# Autodesk Inventor assembly: MeasurementChamber V2 - Assembly - Bade
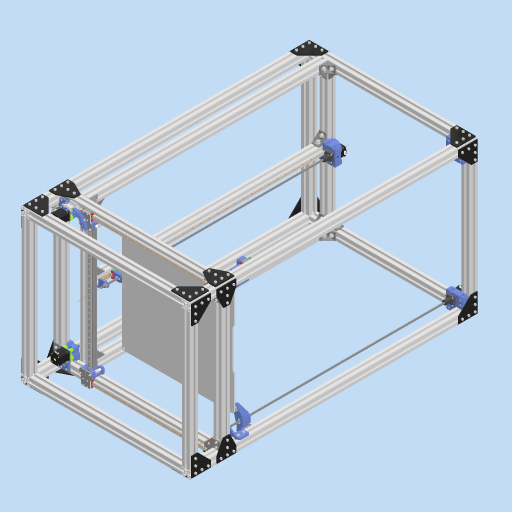
[picture p0: Inventor's stored thumbnail of the model, 512x512]
Saved by Autodesk Inventor 2023.2 (Build 272271000, 271)
## iProperties
Created: 2023-11-28
Part Number: MeasurementChamber V2 - Assembly - Bade
Document SubType Name: Assembly
Designer: Nils Bade
Author: Nils Bade
## Documents named in this file (30)
- C:\Users\nilsb\Documents\Inventor\Projektarbeit-Bade\RatRig_Bade\MeasurementChamber V2 - Assembly - Bade.iam
- C:\Users\nilsb\Documents\Inventor\Projektarbeit-Bade\RatRig_Bade\Z-Axis Transmission Assembly Back.iam
- C:\Users\nilsb\Documents\Inventor\Projektarbeit-Bade\RatRig_Bade\Z-Axis Transmission Assembly Front.iam
- C:\Users\nilsb\Documents\Inventor\Projektarbeit-Bade\RatRig_modified\Lead Screw - TR8x8-2p 1057mm Simple.ipt
- C:\Users\nilsb\Documents\Inventor\Projektarbeit-Bade\RatRig_modified\Leadscrew Constraint Front for 4040 - Assembly.iam
- C:\Users\nilsb\Documents\Inventor\Projektarbeit-Bade\RatRig_modified\Leadscrew Constraint Rear for 4040 - Assembly.iam
- C:\Users\nilsb\Documents\Inventor\Projektarbeit-Bade\RatRig_Bade\Bed Arm Back for 4040 - Assembly.iam
- C:\Users\nilsb\Documents\Inventor\Projektarbeit-Bade\RatRig_Bade\Bed Arm Left for 4040 - Assembly.iam
- C:\Users\nilsb\Documents\Inventor\Projektarbeit-Bade\RatRig_Bade\Bed Arm Right for 4040 - Assembly.iam
- C:\Users\nilsb\Documents\Inventor\Projektarbeit-Bade\RatRig_Bade\CoreXY Idler 4040 Assembly Left.iam
- C:\Users\nilsb\Documents\Inventor\Projektarbeit-Bade\RatRig_Bade\CoreXY Idler 4040 Assembly Right.iam
- C:\Users\nilsb\Documents\Inventor\Projektarbeit-Bade\RatRig_Bade\y-Max Endstop for 4040 - Assembly.iam
- C:\Users\nilsb\Documents\Inventor\Projektarbeit-Bade\Enclosure\enc-SidePanel Unten - Assembly no Absorber.iam
- C:\Users\nilsb\Documents\Inventor\Projektarbeit-Bade\Enclosure\enc-SidePanel Mitte - Assembly no Absorber.iam
- C:\Users\nilsb\Documents\Inventor\Projektarbeit-Bade\Enclosure\enc-SidePanel Oben Links - Assembly no Absorber.iam
- C:\Users\nilsb\Documents\Inventor\Projektarbeit-Bade\Enclosure\enc-SidePanel Oben Rechts - Assembly no Absorber.iam
- C:\Users\nilsb\Documents\Inventor\Projektarbeit-Bade\Enclosure\enc-FrontPanel Oben - Assembly no Absorber.iam
- C:\Users\nilsb\Documents\Inventor\Projektarbeit-Bade\Enclosure\enc-TopPanel - Assembly no Absorber.iam
- C:\Users\nilsb\Documents\Inventor\Projektarbeit-Bade\Enclosure\enc-BackPanel Top - Assembly.iam
- C:\Users\nilsb\Documents\Inventor\Projektarbeit-Bade\Enclosure\enc-BackPanel Unten - Assembly.iam
- C:\Users\nilsb\Documents\Inventor\Projektarbeit-Bade\Enclosure\enc-BackPanel MitteRechts - Assembly.iam
- C:\Users\nilsb\Documents\Inventor\Projektarbeit-Bade\Enclosure\enc-BackPanel MitteLinks - Assembly.iam
- C:\Users\nilsb\Documents\Inventor\Projektarbeit-Bade\Enclosure\enc-BottomPanel.ipt
- C:\Users\nilsb\Documents\Inventor\Projektarbeit-Bade\RatRig_Bade\RatRig-Bade-BedAssembly.iam
- C:\Users\nilsb\Documents\Inventor\Projektarbeit-Bade\RatRig_Bade\MeasurementChamber Frame Assembly - Bade v3.iam
- MeasurementChamber Frame Assembly - Bade v3.iam
- C:\Users\nilsb\Documents\Inventor\Projektarbeit-Bade\RatRig_Bade\X-Gantry Assembly for 4040 V2.iam
- X-Gantry Assembly for 4040 V2.iam
- C:\Users\nilsb\Documents\Inventor\Projektarbeit-Bade\RatRig_Bade\CoreXY Motor Assembly Left for 4040 - V2.iam
- C:\Users\nilsb\Documents\Inventor\Projektarbeit-Bade\RatRig_Bade\CoreXY Motor Assembly Right for 4040 - V2.iam
## Components (36 placed, 26 different names)
1. MeasurementChamber Frame Assembly - Bade v3:1 [sub-assembly] — Passend:85, Passend:86, Passend:87, Passend:88, Passend:89, Passend:90, Passend:91, Passend:92, Passend:93, Passend:94, Passend:95, Passend:96, Passend:97, Passend:98, Passend:99
2. Z-Axis Transmission Assembly Back:1 [sub-assembly] — Passend:13
3. Z-Axis Transmission Assembly Front:1 [sub-assembly] — Passend:15
4. Z-Axis Transmission Assembly Front:2 [sub-assembly] — Passend:14
5. LeadScrew - TR8x8-2p 1057mm Simple:1 — Passend:13
6. LeadScrew - TR8x8-2p 1057mm Simple:2 — Passend:15
7. LeadScrew - TR8x8-2p 1057mm Simple:3 — Passend:14
8. Leadscrew Constraint Front for 4040 - Assembly:1 [sub-assembly] — Fluchtend:22, Fluchtend:1
9. Leadscrew Constraint Front for 4040 - Assembly:2 [sub-assembly] — Fluchtend:22
10. Leadscrew Constraint Rear for 4040 - Assembly:1 [sub-assembly] — Fluchtend:1
11. Bed Arm Back for 4040 - Assembly:1 [sub-assembly] — Fluchtend:29
12. Bed Arm Left for 4040 - Assembly:1 [sub-assembly] — Fluchtend:24, Fluchtend:29
13. Bed Arm Right for 4040 - Assembly:1 [sub-assembly] — Fluchtend:24, Passend:78
14. CoreXY Idler 4040 Assembly Left:1 [sub-assembly] — Passend:89, Passend:90, Passend:91
15. CoreXY Idler 4040 Assembly Right:1 [sub-assembly] — Passend:88, Passend:92, Passend:93
16. CoreXY Motor Assembly Right for 4040:1 [sub-assembly] — Passend:94, Passend:95, Passend:96
17. CoreXY Motor Assembly Left for 4040:1 [sub-assembly] — Passend:97, Passend:98, Passend:99
18. y-Max Endstop for 4040 - Assembly:1 [sub-assembly]
19. enc-SidePanel Unten - Assembly no Absorber:1 [sub-assembly]
20. enc-SidePanel Mitte - Assembly no Absorber:1 [sub-assembly] — Passend:47
21. enc-SidePanel Oben Links - Assembly no Absorber:1 [sub-assembly]
22. enc-SidePanel Unten - Assembly no Absorber:2 [sub-assembly] — Passend:51
23. enc-SidePanel Mitte - Assembly no Absorber:2 [sub-assembly] — Passend:51
24. enc-SidePanel Oben Links- Assembly no Absorber:1 [sub-assembly]
25. enc-SidePanel Unten - Assembly no Absorber:3 [sub-assembly] — Passend:54
26. enc-SidePanel Mitte - Assembly no Absorber:3 [sub-assembly] — Passend:54
27. enc-SidePanel Oben Links - Assembly no Absorber:2 [sub-assembly]
28. enc-TopPanel - Assembly no Absorber:1 [sub-assembly]
29. enc-BackPanel Top - Assembly:1 [sub-assembly]
30. enc-BackPanel Unten - Assembly:1 [sub-assembly]
31. enc-BackPanel Unten - Assembly:2 [sub-assembly]
32. enc-BackPanel MitteRechts- Assembly:1 [sub-assembly]
33. enc-BackPanel MitteLinks - Assembly:1 [sub-assembly]
34. enc-BottomPanel:1
35. RatRig-Bade-BedAssembly:1 [sub-assembly] — Passend:78
36. X-Gantry Assembly for 4040 V2:1 [sub-assembly] — Passend:85, Passend:86, Passend:87
## Relationships (106: Mate 77, Flush 29)
- [Mate]: MeasurementChamber Frame Assembly - Bade v3:1 ↔ Z-Axis Transmission Assembly Back:1
- [Mate]: MeasurementChamber Frame Assembly - Bade v3:1 ↔ Z-Axis Transmission Assembly Back:1
- [Mate]: MeasurementChamber Frame Assembly - Bade v3:1 ↔ Z-Axis Transmission Assembly Back:1
- [Mate]: MeasurementChamber Frame Assembly - Bade v3:1 ↔ Z-Axis Transmission Assembly Front:1
- [Mate]: MeasurementChamber Frame Assembly - Bade v3:1 ↔ Z-Axis Transmission Assembly Front:2
- [Mate]: MeasurementChamber Frame Assembly - Bade v3:1 ↔ Z-Axis Transmission Assembly Front:2
- [Mate]: MeasurementChamber Frame Assembly - Bade v3:1 ↔ Z-Axis Transmission Assembly Front:2
- [Mate]: MeasurementChamber Frame Assembly - Bade v3:1 ↔ Z-Axis Transmission Assembly Front:1
- [Mate]: MeasurementChamber Frame Assembly - Bade v3:1 ↔ Z-Axis Transmission Assembly Front:1
- [Mate]: MeasurementChamber Frame Assembly - Bade v3:1 ↔ LeadScrew - TR8x8-2p 1057mm Simple:1
- [Mate]: MeasurementChamber Frame Assembly - Bade v3:1 ↔ LeadScrew - TR8x8-2p 1057mm Simple:2
- [Mate]: MeasurementChamber Frame Assembly - Bade v3:1 ↔ LeadScrew - TR8x8-2p 1057mm Simple:3
- Passend:13 [Mate] (-10 mm): Z-Axis Transmission Assembly Back:1 ↔ LeadScrew - TR8x8-2p 1057mm Simple:1
- Passend:14 [Mate] (-10 mm): Z-Axis Transmission Assembly Front:2 ↔ LeadScrew - TR8x8-2p 1057mm Simple:3
- Passend:15 [Mate] (-10 mm): Z-Axis Transmission Assembly Front:1 ↔ LeadScrew - TR8x8-2p 1057mm Simple:2
- [Mate]: MeasurementChamber Frame Assembly - Bade v3:1 ↔ Leadscrew Constraint Front for 4040 - Assembly:2
- [Mate]: MeasurementChamber Frame Assembly - Bade v3:1 ↔ Leadscrew Constraint Front for 4040 - Assembly:2
- [Mate] (5 mm): MeasurementChamber Frame Assembly - Bade v3:1 ↔ Leadscrew Constraint Front for 4040 - Assembly:2
- [Mate]: MeasurementChamber Frame Assembly - Bade v3:1 ↔ Leadscrew Constraint Front for 4040 - Assembly:1
- [Mate]: MeasurementChamber Frame Assembly - Bade v3:1 ↔ Leadscrew Constraint Front for 4040 - Assembly:1
- Fluchtend:22 [Flush]: Leadscrew Constraint Front for 4040 - Assembly:1 ↔ Leadscrew Constraint Front for 4040 - Assembly:2
- [Mate]: MeasurementChamber Frame Assembly - Bade v3:1 ↔ Leadscrew Constraint Rear for 4040 - Assembly:1
- [Mate]: MeasurementChamber Frame Assembly - Bade v3:1 ↔ Leadscrew Constraint Rear for 4040 - Assembly:1
- Fluchtend:1 [Flush]: Leadscrew Constraint Front for 4040 - Assembly:1 ↔ Leadscrew Constraint Rear for 4040 - Assembly:1
- [Mate]: MeasurementChamber Frame Assembly - Bade v3:1 ↔ Bed Arm Back for 4040 - Assembly:1
- [Mate]: MeasurementChamber Frame Assembly - Bade v3:1 ↔ Bed Arm Back for 4040 - Assembly:1
- [Flush]: MeasurementChamber Frame Assembly - Bade v3:1 ↔ Bed Arm Left for 4040 - Assembly:1
- [Mate]: MeasurementChamber Frame Assembly - Bade v3:1 ↔ Bed Arm Left for 4040 - Assembly:1
- [Mate]: MeasurementChamber Frame Assembly - Bade v3:1 ↔ Bed Arm Right for 4040 - Assembly:1
- [Mate]: MeasurementChamber Frame Assembly - Bade v3:1 ↔ Bed Arm Right for 4040 - Assembly:1
- Fluchtend:24 [Flush]: Bed Arm Left for 4040 - Assembly:1 ↔ Bed Arm Right for 4040 - Assembly:1
- [Mate]: MeasurementChamber Frame Assembly - Bade v3:1 ↔ y-Max Endstop for 4040 - Assembly:1
- [Mate]: MeasurementChamber Frame Assembly - Bade v3:1 ↔ y-Max Endstop for 4040 - Assembly:1
- Fluchtend:26 [Flush] (135.5 mm)
- Fluchtend:28 [Flush] (1064.95 mm)
- Fluchtend:29 [Flush]: Bed Arm Back for 4040 - Assembly:1 ↔ Bed Arm Left for 4040 - Assembly:1
- Fluchtend:30 [Flush] (1000 mm)
- Fluchtend:31 [Flush] (500 mm)
- [Flush]: MeasurementChamber Frame Assembly - Bade v3:1 ↔ enc-SidePanel Unten - Assembly no Absorber:1
- [Flush]: MeasurementChamber Frame Assembly - Bade v3:1 ↔ enc-SidePanel Unten - Assembly no Absorber:1
- [Mate]: MeasurementChamber Frame Assembly - Bade v3:1 ↔ enc-SidePanel Unten - Assembly no Absorber:1
- [Flush]: MeasurementChamber Frame Assembly - Bade v3:1 ↔ enc-SidePanel Mitte - Assembly no Absorber:1
- Passend:47 [Mate]: enc-SidePanel Mitte - Assembly no Absorber:1
- [Mate]: MeasurementChamber Frame Assembly - Bade v3:1 ↔ enc-SidePanel Mitte - Assembly no Absorber:1
- [Flush]: MeasurementChamber Frame Assembly - Bade v3:1 ↔ enc-SidePanel Oben Links - Assembly no Absorber:1
- [Flush]: MeasurementChamber Frame Assembly - Bade v3:1 ↔ enc-SidePanel Oben Links - Assembly no Absorber:1
- [Mate]: MeasurementChamber Frame Assembly - Bade v3:1 ↔ enc-SidePanel Oben Links - Assembly no Absorber:1
- [Flush]: MeasurementChamber Frame Assembly - Bade v3:1 ↔ enc-SidePanel Unten - Assembly no Absorber:2
- [Flush]: MeasurementChamber Frame Assembly - Bade v3:1 ↔ enc-SidePanel Unten - Assembly no Absorber:2
- [Mate]: MeasurementChamber Frame Assembly - Bade v3:1 ↔ enc-SidePanel Unten - Assembly no Absorber:2
- [Flush]: MeasurementChamber Frame Assembly - Bade v3:1 ↔ enc-SidePanel Mitte - Assembly no Absorber:2
- Passend:51 [Mate]: enc-SidePanel Unten - Assembly no Absorber:2 ↔ enc-SidePanel Mitte - Assembly no Absorber:2
- [Mate]: MeasurementChamber Frame Assembly - Bade v3:1 ↔ enc-SidePanel Mitte - Assembly no Absorber:2
- [Flush]: MeasurementChamber Frame Assembly - Bade v3:1 ↔ enc-SidePanel Oben Links- Assembly no Absorber:1
- [Flush]: MeasurementChamber Frame Assembly - Bade v3:1 ↔ enc-SidePanel Oben Links- Assembly no Absorber:1
- [Mate]: MeasurementChamber Frame Assembly - Bade v3:1 ↔ enc-SidePanel Oben Links- Assembly no Absorber:1
- [Flush]: MeasurementChamber Frame Assembly - Bade v3:1 ↔ enc-SidePanel Unten - Assembly no Absorber:3
- [Flush]: MeasurementChamber Frame Assembly - Bade v3:1 ↔ enc-SidePanel Unten - Assembly no Absorber:3
- [Flush]: MeasurementChamber Frame Assembly - Bade v3:1 ↔ enc-SidePanel Mitte - Assembly no Absorber:3
- Passend:54 [Mate]: enc-SidePanel Unten - Assembly no Absorber:3 ↔ enc-SidePanel Mitte - Assembly no Absorber:3
- [Mate]: MeasurementChamber Frame Assembly - Bade v3:1 ↔ enc-SidePanel Mitte - Assembly no Absorber:3
- [Mate]: MeasurementChamber Frame Assembly - Bade v3:1 ↔ enc-SidePanel Unten - Assembly no Absorber:3
- [Flush]: MeasurementChamber Frame Assembly - Bade v3:1 ↔ enc-SidePanel Oben Links - Assembly no Absorber:2
- [Flush]: MeasurementChamber Frame Assembly - Bade v3:1 ↔ enc-SidePanel Oben Links - Assembly no Absorber:2
- [Mate]: MeasurementChamber Frame Assembly - Bade v3:1 ↔ enc-SidePanel Oben Links - Assembly no Absorber:2
- [Mate]: MeasurementChamber Frame Assembly - Bade v3:1 ↔ enc-TopPanel - Assembly no Absorber:1
- [Mate]: MeasurementChamber Frame Assembly - Bade v3:1 ↔ enc-TopPanel - Assembly no Absorber:1
- [Flush] (5 mm): MeasurementChamber Frame Assembly - Bade v3:1 ↔ enc-TopPanel - Assembly no Absorber:1
- [Mate]: MeasurementChamber Frame Assembly - Bade v3:1 ↔ enc-TopPanel - Assembly no Absorber:1
- [Flush]: MeasurementChamber Frame Assembly - Bade v3:1 ↔ enc-BackPanel Top - Assembly:1
- [Mate]: MeasurementChamber Frame Assembly - Bade v3:1 ↔ enc-BackPanel Top - Assembly:1
- [Mate]: MeasurementChamber Frame Assembly - Bade v3:1 ↔ enc-BackPanel Top - Assembly:1
- [Mate]: MeasurementChamber Frame Assembly - Bade v3:1 ↔ enc-BackPanel Top - Assembly:1
- [Mate]: MeasurementChamber Frame Assembly - Bade v3:1 ↔ enc-BackPanel Unten - Assembly:1
- [Mate]: MeasurementChamber Frame Assembly - Bade v3:1 ↔ enc-BackPanel Unten - Assembly:1
- [Mate]: MeasurementChamber Frame Assembly - Bade v3:1 ↔ enc-BackPanel Unten - Assembly:2
- [Mate]: MeasurementChamber Frame Assembly - Bade v3:1 ↔ enc-BackPanel Unten - Assembly:2
- [Mate]: MeasurementChamber Frame Assembly - Bade v3:1 ↔ enc-BackPanel MitteLinks - Assembly:1
- [Mate]: MeasurementChamber Frame Assembly - Bade v3:1 ↔ enc-BackPanel MitteLinks - Assembly:1
- [Mate]: MeasurementChamber Frame Assembly - Bade v3:1 ↔ enc-BackPanel MitteRechts- Assembly:1
- [Mate]: MeasurementChamber Frame Assembly - Bade v3:1 ↔ enc-BackPanel MitteRechts- Assembly:1
- [Mate]: MeasurementChamber Frame Assembly - Bade v3:1 ↔ enc-BackPanel Unten - Assembly:1
- [Mate]: MeasurementChamber Frame Assembly - Bade v3:1 ↔ enc-BackPanel Unten - Assembly:2
- [Mate]: MeasurementChamber Frame Assembly - Bade v3:1 ↔ enc-BackPanel MitteRechts- Assembly:1
- [Mate]: MeasurementChamber Frame Assembly - Bade v3:1 ↔ enc-BackPanel MitteLinks - Assembly:1
- [Mate]: MeasurementChamber Frame Assembly - Bade v3:1 ↔ enc-BottomPanel:1
- [Flush]: MeasurementChamber Frame Assembly - Bade v3:1 ↔ enc-BottomPanel:1
- [Mate]: MeasurementChamber Frame Assembly - Bade v3:1 ↔ enc-BottomPanel:1
- [Flush]: MeasurementChamber Frame Assembly - Bade v3:1 ↔ RatRig-Bade-BedAssembly:1
- Passend:78 [Mate] (18 mm): Bed Arm Right for 4040 - Assembly:1 ↔ RatRig-Bade-BedAssembly:1
- [Flush] (-327 mm): MeasurementChamber Frame Assembly - Bade v3:1 ↔ RatRig-Bade-BedAssembly:1
- Passend:85 [Mate]: MeasurementChamber Frame Assembly - Bade v3:1 ↔ X-Gantry Assembly for 4040 V2:1
- Passend:86 [Mate]: MeasurementChamber Frame Assembly - Bade v3:1 ↔ X-Gantry Assembly for 4040 V2:1
- Passend:87 [Mate]: MeasurementChamber Frame Assembly - Bade v3:1 ↔ X-Gantry Assembly for 4040 V2:1
- Passend:88 [Mate]: MeasurementChamber Frame Assembly - Bade v3:1 ↔ CoreXY Idler 4040 Assembly Right:1
- Passend:89 [Mate]: MeasurementChamber Frame Assembly - Bade v3:1 ↔ CoreXY Idler 4040 Assembly Left:1
- Passend:90 [Mate]: MeasurementChamber Frame Assembly - Bade v3:1 ↔ CoreXY Idler 4040 Assembly Left:1
- Passend:91 [Mate]: MeasurementChamber Frame Assembly - Bade v3:1 ↔ CoreXY Idler 4040 Assembly Left:1
- Passend:92 [Mate]: MeasurementChamber Frame Assembly - Bade v3:1 ↔ CoreXY Idler 4040 Assembly Right:1
- Passend:93 [Mate]: MeasurementChamber Frame Assembly - Bade v3:1 ↔ CoreXY Idler 4040 Assembly Right:1
- Passend:94 [Mate]: MeasurementChamber Frame Assembly - Bade v3:1 ↔ CoreXY Motor Assembly Right for 4040:1
- Passend:95 [Mate]: MeasurementChamber Frame Assembly - Bade v3:1 ↔ CoreXY Motor Assembly Right for 4040:1
- Passend:96 [Mate]: MeasurementChamber Frame Assembly - Bade v3:1 ↔ CoreXY Motor Assembly Right for 4040:1
- Passend:97 [Mate]: MeasurementChamber Frame Assembly - Bade v3:1 ↔ CoreXY Motor Assembly Left for 4040:1
- Passend:98 [Mate]: MeasurementChamber Frame Assembly - Bade v3:1 ↔ CoreXY Motor Assembly Left for 4040:1
- Passend:99 [Mate]: MeasurementChamber Frame Assembly - Bade v3:1 ↔ CoreXY Motor Assembly Left for 4040:1
